# Autodesk Inventor assembly: Tuer_MIR
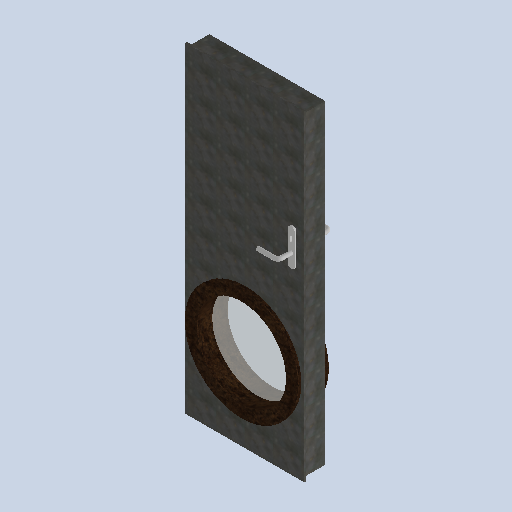
[picture p0: Inventor's stored thumbnail of the model, 512x512]
Saved by Autodesk Inventor 2025.1 (Build 291241000, 241)
## iProperties
Created: 2024-08-07
Part Number: Tuer_MIR
Document SubType Name: Assembly
Designer: ffogue
Author: ffogue
## Documents named in this file (6)
- C:\Users\ffogue\Documents\Inventor\BrandschutzTuer\Tuer_MIR.iam
- C:\Users\ffogue\Documents\Inventor\BrandschutzTuer\Rahmen_MIR.ipt
- C:\Users\ffogue\Documents\Inventor\BrandschutzTuer\Schutz_MIR.ipt
- C:\Users\ffogue\Documents\Inventor\BrandschutzTuer\garnitur_lang_MIR.ipt
- C:\Users\ffogue\Documents\Inventor\BrandschutzTuer\garnitur_lang_links_MIR.ipt
- C:\Users\ffogue\Documents\Inventor\BrandschutzTuer\glassMitSchutz_MIR.iam
## Components (5 placed, 5 different names)
1. Rahmen_MIR:1 — Flush:4, Flush:3, Flush:2, Insert:1, Mate:2, Mate:1
2. Schutz_MIR:1 — Flush:4, Flush:3, Flush:2, Insert:2, Mate:4, Mate:3, Insert:3
3. garnitur_lang_MIR:1 — Insert:1, Mate:2, Mate:1
4. garnitur_lang_links_MIR:1 — Insert:2, Mate:4, Mate:3
5. glassMitSchutz_MIR:1 [sub-assembly] — Insert:3
## Relationships (10: Mate 4, Flush 3, Insert 3)
- Flush:4 (65 mm): Rahmen_MIR:1 ↔ Schutz_MIR:1
- Flush:3 (19 mm): Rahmen_MIR:1 ↔ Schutz_MIR:1
- Flush:2 (9.5 mm): Rahmen_MIR:1 ↔ Schutz_MIR:1
- Insert:1: Rahmen_MIR:1 ↔ garnitur_lang_MIR:1
- Mate:2: Rahmen_MIR:1 ↔ garnitur_lang_MIR:1
- Mate:1: Rahmen_MIR:1 ↔ garnitur_lang_MIR:1
- Insert:2: Schutz_MIR:1 ↔ garnitur_lang_links_MIR:1
- Mate:4: Schutz_MIR:1 ↔ garnitur_lang_links_MIR:1
- Mate:3: Schutz_MIR:1 ↔ garnitur_lang_links_MIR:1
- Insert:3: Schutz_MIR:1 ↔ glassMitSchutz_MIR:1
